# Autodesk Inventor assembly: Medical Air Filter Assy (1)
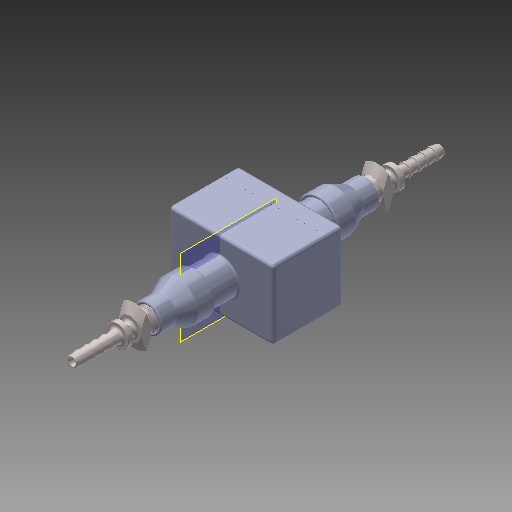
[picture p0: Inventor's stored thumbnail of the model, 512x512]
Saved by Autodesk Inventor 2018 (Build 220112000, 112)
## iProperties
Created: 2020-03-31
Part Number: Medical Air Filter Assy (1)
Description: STEP AP214
Document SubType Name: Assembly
Designer: emile
Sending System: SolidWorks 2017
Preprocessor: SwSTEP 2.0
Title: Medical Air Filter Assy.STEP
Revision Number: ANY
## Documents named in this file (6)
- C:\Users\emile\OneDrive\Documents\GitHub\VentilatorCovid19\Respirator\MultiLine\MedicalAirFilter\Medical Air Filter Assy (1).iam
- C:\Users\emile\OneDrive\Documents\GitHub\VentilatorCovid19\Respirator\MultiLine\MedicalAirFilter\Medical Air Filter Bottom.ipt
- C:\Users\emile\OneDrive\Documents\GitHub\VentilatorCovid19\Respirator\MultiLine\MedicalAirFilter\Medical Air Filter Top.ipt
- C:\Users\emile\OneDrive\Documents\GitHub\VentilatorCovid19\Respirator\MultiLine\MedicalAirFilter\Medical Air Filter.ipt
- C:\Users\emile\OneDrive\Documents\GitHub\VentilatorCovid19\Respirator\MultiLine\MedicalAirFilter\22mm to 0.25 inch pipe adapter.ipt
- C:\Users\emile\OneDrive\Documents\GitHub\VentilatorCovid19\Respirator\MultiLine\MedicalAirFilter\Vanamatic-4130.ipt
## Components (7 placed, 7 different names)
1. Medical Air Filter Bottom_1 — Symmetry:1
2. Medical Air Filter Top_2
3. Medical Air Filter_3 — Symmetry:1
4. 22mm to 0.25 inch pipe adapter_4
5. 22mm to 0.25 inch pipe adapter_5
6. Vanamatic-4130_6
7. Vanamatic-4130_7
## Relationships (1: Symmetry 1)
- Symmetry:1: Medical Air Filter Bottom_1 ↔ Medical Air Filter_3
